# Autodesk Inventor assembly: mini Cryostat FOOT3
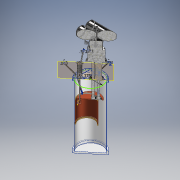
[picture p0: Inventor's stored thumbnail of the model, 180x180]
Saved by Autodesk Inventor 2018 (Build 220112000, 112)
## iProperties
Created: 2018-10-10
Part Number: mini Cryostat FOOT3
Document SubType Name: Assembly
Designer: Admin
Author: Admin
## Documents named in this file (12)
- C:\Users\Admin\Documents\Cryostat\CAD\mini Cryostat FOOT3.iam
- C:\Users\Admin\Documents\Cryostat\CAD\External Models\CH40415 24JUL14 C.ipt
- C:\Users\Admin\Documents\Cryostat\CAD\vacuum jacket long.ipt
- C:\Users\Admin\Documents\Cryostat\CAD\vacuum jacket.ipt
- C:\Users\Admin\Documents\Cryostat\CAD\Top Plate V2.2.ipt
- C:\Users\Admin\Documents\Cryostat\CAD\mini 55K stage.ipt
- C:\Users\Admin\Documents\Cryostat\CAD\foot type 3.iam
- C:\Users\Admin\Documents\Cryostat\CAD\2K8 stage mini.ipt
- C:\Users\Admin\Documents\Cryostat\CAD\Radiation Sheild 2K.ipt
- C:\Users\Admin\Documents\Cryostat\CAD\2K8 FEET.iam
- C:\Users\Admin\Documents\Cryostat\CAD\still pipe.iam
- C:\Users\Admin\Documents\Cryostat\CAD\4K shield.iam
## Components (21 placed, 11 different names)
1. Top Plate V2.2:1 — Mate:16, Mate:18, Mate:19, Mate:20, Mate:21, Mate:26, Mate:135, Mate:136, Mate:137, Mate:138, Mate:139, Mate:140, Mate:141, Mate:142, Mate:143, Mate:144, Mate:145, Mate:146, Mate:149, Mate:150, Mate:153, Mate:154, Mate:155, Mate:156
2. CH40415 24JUL14 C:1 — Mate:16, Mate:18, Mate:26, Mate:161
3. vacuum jacket long:1 — Mate:7, Mate:8, Mate:9
4. vacuum jacket:1 — Mate:7, Mate:8, Mate:9, Mate:19, Mate:20, Mate:21
5. mini 55K stage:1 — Mate:100, Mate:102, Mate:107, Mate:108, Mate:109, Mate:110, Mate:111, Mate:112, Mate:113, Mate:114, Mate:147, Mate:148, Mate:151, Mate:152, Mate:157, Mate:158, Mate:159, Mate:160, Mate:161, Mate:162, Mate:163, Mate:164, Mate:165, Mate:166, Mate:167, Mate:168, Mate:169, Mate:170, Mate:172
6. 2K8 stage mini:1 — Mate:125, Mate:126, Mate:127, Mate:128, Mate:129, Mate:130, Mate:131, Mate:132
7. Radiation Sheild 2K:1 — Mate:100, Mate:102
8. 2K8 FEET:1 [sub-assembly] — Mate:107, Mate:108, Mate:127, Mate:131
9. 2K8 FEET:2 [sub-assembly] — Mate:109, Mate:113, Mate:128, Mate:132
10. 2K8 FEET:3 [sub-assembly] — Mate:110, Mate:112, Mate:125, Mate:129
11. 2K8 FEET:4 [sub-assembly] — Mate:111, Mate:114, Mate:126, Mate:130
12. still pipe:1 [sub-assembly] — Mate:135, Mate:136, Mate:162, Mate:172
13. foot type 3:1 [sub-assembly] — Mate:143, Mate:155, Mate:158, Mate:164
14. foot type 3:2 [sub-assembly] — Mate:140, Mate:153, Mate:159, Mate:169, Mate:173
15. foot type 3:3 [sub-assembly] — Mate:138, Mate:149, Mate:151, Mate:163
16. foot type 3:4 [sub-assembly] — Mate:144, Mate:154, Mate:160, Mate:168
17. foot type 3:5 [sub-assembly] — Mate:139, Mate:150, Mate:152, Mate:170
18. foot type 3:6 [sub-assembly] — Mate:137, Mate:145, Mate:148, Mate:166
19. foot type 3:7 [sub-assembly] — Mate:141, Mate:156, Mate:157, Mate:165, Mate:174
20. foot type 3:8 [sub-assembly] — Mate:142, Mate:146, Mate:147, Mate:167
21. 4K shield:1 [sub-assembly]
## Relationships (66: Mate 66)
- Mate:7: vacuum jacket long:1 ↔ vacuum jacket:1
- Mate:8: vacuum jacket long:1 ↔ vacuum jacket:1
- Mate:9: vacuum jacket long:1 ↔ vacuum jacket:1
- Mate:16: Top Plate V2.2:1 ↔ CH40415 24JUL14 C:1
- Mate:18: Top Plate V2.2:1 ↔ CH40415 24JUL14 C:1
- Mate:19: Top Plate V2.2:1 ↔ vacuum jacket:1
- Mate:20: Top Plate V2.2:1 ↔ vacuum jacket:1
- Mate:21: Top Plate V2.2:1 ↔ vacuum jacket:1
- Mate:26: Top Plate V2.2:1 ↔ CH40415 24JUL14 C:1
- Mate:100: mini 55K stage:1 ↔ Radiation Sheild 2K:1
- Mate:102: mini 55K stage:1 ↔ Radiation Sheild 2K:1
- Mate:107: mini 55K stage:1 ↔ 2K8 FEET:1
- Mate:108: mini 55K stage:1 ↔ 2K8 FEET:1
- Mate:109: mini 55K stage:1 ↔ 2K8 FEET:2
- Mate:110: mini 55K stage:1 ↔ 2K8 FEET:3
- Mate:111: mini 55K stage:1 ↔ 2K8 FEET:4
- Mate:112: mini 55K stage:1 ↔ 2K8 FEET:3
- Mate:113: mini 55K stage:1 ↔ 2K8 FEET:2
- Mate:114: mini 55K stage:1 ↔ 2K8 FEET:4
- Mate:125: 2K8 stage mini:1 ↔ 2K8 FEET:3
- Mate:126: 2K8 stage mini:1 ↔ 2K8 FEET:4
- Mate:127: 2K8 stage mini:1 ↔ 2K8 FEET:1
- Mate:128: 2K8 stage mini:1 ↔ 2K8 FEET:2
- Mate:129: 2K8 stage mini:1 ↔ 2K8 FEET:3
- Mate:130: 2K8 stage mini:1 ↔ 2K8 FEET:4
- Mate:131: 2K8 stage mini:1 ↔ 2K8 FEET:1
- Mate:132: 2K8 stage mini:1 ↔ 2K8 FEET:2
- Mate:135: Top Plate V2.2:1 ↔ still pipe:1
- Mate:136: Top Plate V2.2:1 ↔ still pipe:1
- Mate:137: Top Plate V2.2:1 ↔ foot type 3:6
- Mate:138: Top Plate V2.2:1 ↔ foot type 3:3
- Mate:139: Top Plate V2.2:1 ↔ foot type 3:5
- Mate:140: Top Plate V2.2:1 ↔ foot type 3:2
- Mate:141: Top Plate V2.2:1 ↔ foot type 3:7
- Mate:142: Top Plate V2.2:1 ↔ foot type 3:8
- Mate:143: Top Plate V2.2:1 ↔ foot type 3:1
- Mate:144: Top Plate V2.2:1 ↔ foot type 3:4
- Mate:145: Top Plate V2.2:1 ↔ foot type 3:6
- Mate:146: Top Plate V2.2:1 ↔ foot type 3:8
- Mate:147: mini 55K stage:1 ↔ foot type 3:8
- Mate:148: mini 55K stage:1 ↔ foot type 3:6
- Mate:149: Top Plate V2.2:1 ↔ foot type 3:3
- Mate:150: Top Plate V2.2:1 ↔ foot type 3:5
- Mate:151: mini 55K stage:1 ↔ foot type 3:3
- Mate:152: mini 55K stage:1 ↔ foot type 3:5
- Mate:153: Top Plate V2.2:1 ↔ foot type 3:2
- Mate:154: Top Plate V2.2:1 ↔ foot type 3:4
- Mate:155: Top Plate V2.2:1 ↔ foot type 3:1
- Mate:156: Top Plate V2.2:1 ↔ foot type 3:7
- Mate:157: mini 55K stage:1 ↔ foot type 3:7
- Mate:158: mini 55K stage:1 ↔ foot type 3:1
- Mate:159: mini 55K stage:1 ↔ foot type 3:2
- Mate:160: mini 55K stage:1 ↔ foot type 3:4
- Mate:161: CH40415 24JUL14 C:1 ↔ mini 55K stage:1
- Mate:162: mini 55K stage:1 ↔ still pipe:1
- Mate:163: mini 55K stage:1 ↔ foot type 3:3
- Mate:164: mini 55K stage:1 ↔ foot type 3:1
- Mate:165: mini 55K stage:1 ↔ foot type 3:7
- Mate:166: mini 55K stage:1 ↔ foot type 3:6
- Mate:167: mini 55K stage:1 ↔ foot type 3:8
- Mate:168: mini 55K stage:1 ↔ foot type 3:4
- Mate:169: mini 55K stage:1 ↔ foot type 3:2
- Mate:170: mini 55K stage:1 ↔ foot type 3:5
- Mate:172: mini 55K stage:1 ↔ still pipe:1
- Mate:173: foot type 3:2
- Mate:174: foot type 3:7
